# Autodesk Inventor assembly: Jetson Nano
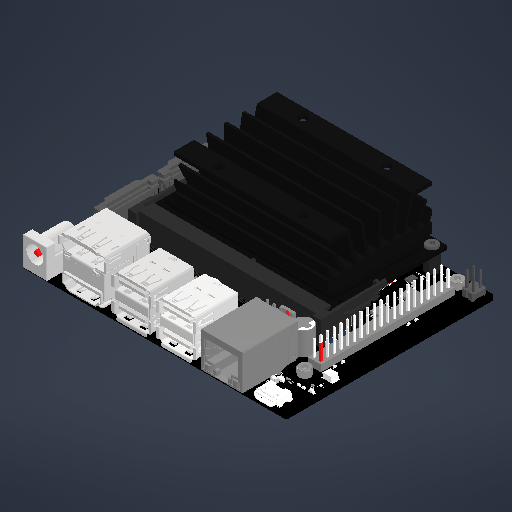
[picture p0: Inventor's stored thumbnail of the model, 512x512]
Saved by Autodesk Inventor 2025.2 (Build 292293000, 293)
## iProperties
Company: .
Created: 2019-05-09
Part Number: Jetson Nano
Document SubType Name: Assembly
Designer: EB
Sending System: CREO PARAMETRIC BY PTC INC, 2018070
Preprocessor: CREO PARAMETRIC BY PTC INC, 2018070
Title: 675-13450_PORG_DEV_KIT_TOP_ASSY
Author: ysung
Revision Number: 1LAST_VERSION
## Documents named in this file (5)
- C:\Users\Faabs\Desktop\TeamFaabs-CAD v2023\OBG\OBG-Jetson Nano.iam
- C:\Users\Faabs\Desktop\TeamFaabs-CAD v2023\OBG\Jetson_Nano_Dev_Kit_3D_b01\642-13450_PORG_SYS_BOM.iam
- C:\Users\Faabs\Desktop\TeamFaabs-CAD v2023\OBG\Jetson_Nano_Dev_Kit_3D_b01\682-13450_PORG_ME_THER_ASSY.iam
- C:\Users\Faabs\Desktop\TeamFaabs-CAD v2023\Verbindungselemente\Abstandsbolzen_Jetson.ipt
- C:\Users\Faabs\Desktop\TeamFaabs-CAD v2023\Verbindungselemente\DIN 912\DIN 912 - M2,5 x 0,45 x 4 x 2,875.ipt
## Components (10 placed, 4 different names)
1. 406 [sub-assembly] — Einfügen:1, Einfügen:2, Einfügen:3, Einfügen:4, Einfügen:5, Einfügen:6, Einfügen:7, Einfügen:8
2. 420 [sub-assembly]
3. Abstandsbolzen_Jetson:1 — Einfügen:2
4. Abstandsbolzen_Jetson:2 — Einfügen:1
5. Abstandsbolzen_Jetson:3 — Einfügen:4
6. Abstandsbolzen_Jetson:4 — Einfügen:3
7. DIN 912 - ersetzt durch DIN EN ISO 4762 M2,5 x 4:1 — Einfügen:7
8. DIN 912 - ersetzt durch DIN EN ISO 4762 M2,5 x 4:2 — Einfügen:8
9. DIN 912 - ersetzt durch DIN EN ISO 4762 M2,5 x 4:3 — Einfügen:6
10. DIN 912 - ersetzt durch DIN EN ISO 4762 M2,5 x 4:4 — Einfügen:5
## Relationships (8: Insert 8)
- Einfügen:1 [Insert]: 406 ↔ Abstandsbolzen_Jetson:2
- Einfügen:2 [Insert]: 406 ↔ Abstandsbolzen_Jetson:1
- Einfügen:3 [Insert]: 406 ↔ Abstandsbolzen_Jetson:4
- Einfügen:4 [Insert]: 406 ↔ Abstandsbolzen_Jetson:3
- Einfügen:5 [Insert]: 406 ↔ DIN 912 - ersetzt durch DIN EN ISO 4762 M2,5 x 4:4
- Einfügen:6 [Insert]: 406 ↔ DIN 912 - ersetzt durch DIN EN ISO 4762 M2,5 x 4:3
- Einfügen:7 [Insert]: 406 ↔ DIN 912 - ersetzt durch DIN EN ISO 4762 M2,5 x 4:1
- Einfügen:8 [Insert]: 406 ↔ DIN 912 - ersetzt durch DIN EN ISO 4762 M2,5 x 4:2
